# Autodesk Inventor assembly: Planetary Gearbox
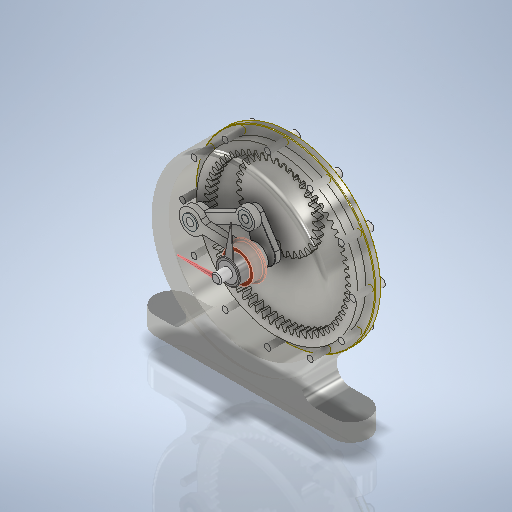
[picture p0: Inventor's stored thumbnail of the model, 512x512]
Saved by Autodesk Inventor 2025.1 (Build 291241000, 241)
## iProperties
Created: 2024-09-02
Part Number: Planetary Gearbox
Document SubType Name: Assembly
Designer: ffogue
Author: ffogue
## Documents named in this file (13)
- C:\Users\ffogue\Documents\Inventor\Planetary Gear\Planetary Gearbox.iam
- C:\Users\ffogue\Documents\Inventor\Planetary Gear\101 part 2.ipt
- C:\Users\ffogue\Documents\Inventor\Planetary Gear\101 part 3.ipt
- C:\Users\ffogue\Documents\Inventor\Planetary Gear\101 part 1.ipt
- C:\Users\ffogue\Documents\Inventor\Planetary Gear\204.ipt
- C:\Users\ffogue\Documents\Inventor\Planetary Gear\203 part 1.ipt
- C:\Users\ffogue\Documents\Inventor\Planetary Gear\203 part 3.ipt
- C:\Users\ffogue\Documents\Inventor\Planetary Gear\204 part 1.ipt
- C:\Users\ffogue\Documents\Inventor\Planetary Gear\Spur Gear21_135.ipt
- C:\Users\ffogue\Documents\Inventor\Planetary Gear\201 part 2.ipt
- C:\Users\ffogue\Documents\Inventor\Planetary Gear\202 part 3.ipt
- C:\Users\ffogue\Documents\Inventor\Planetary Gear\201 part 1 gear.ipt
- C:\Users\ffogue\Documents\Inventor\Planetary Gear\fastener.ipt
## Components (24 placed, 12 different names)
1. 101 part 2:1 — Mate:1, Insert:1, Mate:3, Insert:3, Mate:9, Flush:4
2. 101 part 3:1 — Mate:1, Insert:1, Mate:4, Insert:4
3. 101 part 1:1 — Mate:3, Insert:3, Mate:15, Insert:9
4. 203 part 1:1 — Mate:4, Insert:4, Mate:5, Mate:6, Flush:1, Mate:8, Flush:3, Mate:10, Rotation:3
5. 204:1 — Mate:5, Mate:7, Insert:5, Insert:6
6. 203 part 3:1 — Mate:6, Flush:1, Insert:7
7. 204 part 1:1 — Mate:7, Insert:6, Mate:12, Insert:8
8. 204 part 1:2 — Mate:8, Flush:3, Insert:5
9. Spur Gear2:1 — Mate:9, Flush:4, Rotation:1, Flush:5, Tangent:1
10. 202 part 3:1 — Mate:10, Insert:7, Mate:13, Rotation:2, Rotation:3, Mate:14
11. 201 part 2:1 — Mate:12, Insert:8, Mate:13
12. Stirnzahnrad1:1 — Angle:3, Rotation:1, Rotation:2, Flush:5, Tangent:1, Mate:14
13. fastener:1 — Mate:15, Insert:9
14. fastener:2
15. fastener:3
16. fastener:4
17. fastener:5
18. fastener:6
19. fastener:7
20. fastener:8
21. fastener:9
22. fastener:10
23. fastener:11
24. fastener:12
## Component patterns: (12 elements, first: fastener:1)
## Relationships (30: Mate 13, Insert 8, Flush 4, RelateRotation 3, Angle 1, Tangent 1)
- Mate:1: 101 part 2:1 ↔ 101 part 3:1
- Insert:1: 101 part 2:1 ↔ 101 part 3:1
- Mate:3: 101 part 2:1 ↔ 101 part 1:1
- Insert:3: 101 part 2:1 ↔ 101 part 1:1
- Mate:4: 101 part 3:1 ↔ 203 part 1:1
- Insert:4 (-18 mm): 101 part 3:1 ↔ 203 part 1:1
- Mate:5: 203 part 1:1 ↔ 204:1
- Mate:6: 203 part 1:1 ↔ 203 part 3:1
- Flush:1: 203 part 1:1 ↔ 203 part 3:1
- Mate:7: 204:1 ↔ 204 part 1:1
- Mate:8: 203 part 1:1 ↔ 204 part 1:2
- Flush:3 (-1 mm): 203 part 1:1 ↔ 204 part 1:2
- Insert:5: 204:1 ↔ 204 part 1:2
- Mate:9: 101 part 2:1 ↔ Spur Gear2:1
- Flush:4: 101 part 2:1 ↔ Spur Gear2:1
- Insert:6 (-6 mm): 204:1 ↔ 204 part 1:1
- Mate:10: 203 part 1:1 ↔ 202 part 3:1
- Insert:7 (-35 mm): 203 part 3:1 ↔ 202 part 3:1
- Mate:12: 204 part 1:1 ↔ 201 part 2:1
- Insert:8: 204 part 1:1 ↔ 201 part 2:1
- Mate:13: 202 part 3:1 ↔ 201 part 2:1
- Angle:3 (360 deg): Stirnzahnrad1:1
- Rotation:1 [RelateRotation] (0.5 ul): Spur Gear2:1 ↔ Stirnzahnrad1:1
- Rotation:2 [RelateRotation] (1 ul): 202 part 3:1 ↔ Stirnzahnrad1:1
- Rotation:3 [RelateRotation] (1 ul): 203 part 1:1 ↔ 202 part 3:1
- Flush:5: Spur Gear2:1 ↔ Stirnzahnrad1:1
- Tangent:1: Spur Gear2:1 ↔ Stirnzahnrad1:1
- Mate:14: 202 part 3:1 ↔ Stirnzahnrad1:1
- Mate:15: 101 part 1:1 ↔ fastener:1
- Insert:9: 101 part 1:1 ↔ fastener:1
